# Autodesk Inventor assembly: tosaerba
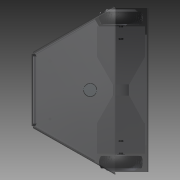
[picture p0: Inventor's stored thumbnail of the model, 180x180]
Saved by Autodesk Inventor 2014 SP2 (Build 180246200, 246)
## iProperties
Created: 2019-04-05
Part Number: tosaerba
Document SubType Name: Assembly
Designer: GauchoHP
Author: GauchoHP
## Documents named in this file (15)
- C:\Users\GauchoHP\Desktop\tosaerba\LawnmowerMechanicalProject\3D PROJECT - INVENTOR 2014\tosaerba.iam
- C:\Users\GauchoHP\Desktop\tosaerba\LawnmowerMechanicalProject\3D PROJECT - INVENTOR 2014\piastra.ipt
- C:\Users\GauchoHP\Desktop\tosaerba\LawnmowerMechanicalProject\3D PROJECT - INVENTOR 2014\motore.iam
- C:\Users\GauchoHP\Desktop\tosaerba\LawnmowerMechanicalProject\3D PROJECT - INVENTOR 2014\Imported Components\ruota pivottante\Assembly15.iam
- C:\Users\GauchoHP\Desktop\tosaerba\LawnmowerMechanicalProject\3D PROJECT - INVENTOR 2014\hoverboard naked.iam
- C:\Users\GauchoHP\Desktop\tosaerba\LawnmowerMechanicalProject\3D PROJECT - INVENTOR 2014\Imported Components\ruota pivottante\Assembly1.iam
- C:\Users\GauchoHP\Desktop\tosaerba\LawnmowerMechanicalProject\3D PROJECT - INVENTOR 2014\coverPolicarbonato2.ipt
- C:\Users\GauchoHP\Desktop\tosaerba\LawnmowerMechanicalProject\3D PROJECT - INVENTOR 2014\sponda laterale policarbonato.ipt
- C:\Users\GauchoHP\Desktop\tosaerba\LawnmowerMechanicalProject\3D PROJECT - INVENTOR 2014\lama\dadoAutobloccante.ipt
- C:\Users\GauchoHP\Desktop\tosaerba\LawnmowerMechanicalProject\3D PROJECT - INVENTOR 2014\lama\vite.ipt
- C:\Users\GauchoHP\Desktop\tosaerba\LawnmowerMechanicalProject\3D PROJECT - INVENTOR 2014\supportoCuscinettoAlto.ipt
- C:\Users\GauchoHP\Desktop\tosaerba\LawnmowerMechanicalProject\3D PROJECT - INVENTOR 2014\lama\bearing.ipt
- C:\Users\GauchoHP\Desktop\tosaerba\LawnmowerMechanicalProject\3D PROJECT - INVENTOR 2014\lama\bladeSupport.ipt
- C:\Users\GauchoHP\Desktop\tosaerba\LawnmowerMechanicalProject\3D PROJECT - INVENTOR 2014\lama\boltCap.ipt
- C:\Users\GauchoHP\Desktop\tosaerba\LawnmowerMechanicalProject\3D PROJECT - INVENTOR 2014\lama\lametta.ipt
## Components (21 placed, 14 different names)
1. piastra:1 — Mate:8, Mate:37, Mate:45, Mate:46, Flush:3, Mate:47, Flush:4, Mate:48, Mate:49, Flush:5, Flush:6, Flush:7, Flush:8, Mate:50, Mate:51, Mate:52, Mate:54, Mate:55, Mate:81, Mate:82, Flush:14
2. motore:1 [sub-assembly] — Mate:8, Mate:84, Flush:14
3. Assembly15:1 [sub-assembly] — Mate:54, Mate:55
4. hoverboard naked:1 [sub-assembly] — Mate:37, Flush:2, Mate:48
5. Assembly1:1 [sub-assembly] — Mate:51, Mate:52
6. coverPolicarbonato2:1 — Flush:2, Mate:45, Mate:46, Flush:4
7. sponda laterale policarbonato:1 — Mate:49, Flush:5, Flush:6
8. sponda laterale policarbonato:2 — Flush:7, Flush:8, Mate:50
9. dadoAutobloccante:1 — Mate:65, Flush:10, Mate:67
10. dadoAutobloccante:2 — Mate:68, Mate:71, Mate:82
11. vite:1 — Mate:61, Mate:62, Mate:63, Mate:65, Mate:66, Mate:68, Mate:69, Mate:83, Mate:84
12. supportoCuscinettoAlto:1 — Mate:57, Flush:9, Mate:63, Mate:64
13. bearing:1 — Mate:57, Flush:9, Mate:62, Mate:83
14. bearing:2 — Mate:59, Mate:60
15. supportoCuscinettoAlto:2 — Mate:59, Mate:60, Mate:61, Mate:64, Flush:10, Mate:81
16. bladeSupport:1 — Mate:66, Mate:67, Mate:70, Mate:72, Mate:73, Mate:74, Flush:11, Mate:75, Mate:76, Flush:12, Mate:77, Mate:78, Flush:13, Mate:79, Mate:80
17. boltCap:1 — Mate:69, Mate:70, Mate:71
18. lametta:1 — Mate:72, Mate:73, Mate:74
19. lametta:2 — Flush:11, Mate:75, Mate:76
20. lametta:3 — Flush:12, Mate:77, Mate:78
21. lametta:4 — Flush:13, Mate:79, Mate:80
## Relationships (52: Mate 39, Flush 13)
- Mate:8: piastra:1 ↔ motore:1
- Mate:37: piastra:1 ↔ hoverboard naked:1
- Flush:2 (5.5 mm): hoverboard naked:1 ↔ coverPolicarbonato2:1
- Mate:45: piastra:1 ↔ coverPolicarbonato2:1
- Mate:46 (20 mm): piastra:1 ↔ coverPolicarbonato2:1
- Flush:3: piastra:1
- Mate:47 (66 mm): piastra:1
- Flush:4 (8 mm): piastra:1 ↔ coverPolicarbonato2:1
- Mate:48 (5 mm): piastra:1 ↔ hoverboard naked:1
- Mate:49: piastra:1 ↔ sponda laterale policarbonato:1
- Flush:5: piastra:1 ↔ sponda laterale policarbonato:1
- Flush:6 (20 mm): piastra:1 ↔ sponda laterale policarbonato:1
- Flush:7: piastra:1 ↔ sponda laterale policarbonato:2
- Flush:8 (-20 mm): piastra:1 ↔ sponda laterale policarbonato:2
- Mate:50: piastra:1 ↔ sponda laterale policarbonato:2
- Mate:51: piastra:1 ↔ Assembly1:1
- Mate:52: piastra:1 ↔ Assembly1:1
- Mate:54: piastra:1 ↔ Assembly15:1
- Mate:55: piastra:1 ↔ Assembly15:1
- Mate:57: supportoCuscinettoAlto:1 ↔ bearing:1
- Mate:59: bearing:2 ↔ supportoCuscinettoAlto:2
- Mate:60: bearing:2 ↔ supportoCuscinettoAlto:2
- Mate:61: vite:1 ↔ supportoCuscinettoAlto:2
- Flush:9: supportoCuscinettoAlto:1 ↔ bearing:1
- Mate:62: vite:1 ↔ bearing:1
- Mate:63 (-3 mm): vite:1 ↔ supportoCuscinettoAlto:1
- Mate:64 (3 mm): supportoCuscinettoAlto:1 ↔ supportoCuscinettoAlto:2
- Mate:65: dadoAutobloccante:1 ↔ vite:1
- Flush:10 (-10 mm): dadoAutobloccante:1 ↔ supportoCuscinettoAlto:2
- Mate:66: vite:1 ↔ bladeSupport:1
- Mate:67: dadoAutobloccante:1 ↔ bladeSupport:1
- Mate:68: dadoAutobloccante:2 ↔ vite:1
- Mate:69: vite:1 ↔ boltCap:1
- Mate:70: bladeSupport:1 ↔ boltCap:1
- Mate:71: dadoAutobloccante:2 ↔ boltCap:1
- Mate:72: bladeSupport:1 ↔ lametta:1
- Mate:73: bladeSupport:1 ↔ lametta:1
- Mate:74: bladeSupport:1 ↔ lametta:1
- Flush:11 (-0.8 mm): bladeSupport:1 ↔ lametta:2
- Mate:75: bladeSupport:1 ↔ lametta:2
- Mate:76: bladeSupport:1 ↔ lametta:2
- Flush:12 (-0.8 mm): bladeSupport:1 ↔ lametta:3
- Mate:77: bladeSupport:1 ↔ lametta:3
- Mate:78: bladeSupport:1 ↔ lametta:3
- Flush:13 (-0.8 mm): bladeSupport:1 ↔ lametta:4
- Mate:79: bladeSupport:1 ↔ lametta:4
- Mate:80: bladeSupport:1 ↔ lametta:4
- Mate:81: piastra:1 ↔ supportoCuscinettoAlto:2
- Mate:82: piastra:1 ↔ dadoAutobloccante:2
- Mate:83: vite:1 ↔ bearing:1
- Mate:84: motore:1 ↔ vite:1
- Flush:14 (15.364 mm): piastra:1 ↔ motore:1
